# Autodesk Inventor assembly: componentes
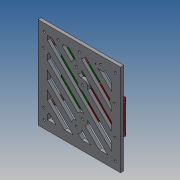
[picture p0: Inventor's stored thumbnail of the model, 180x180]
Saved by Autodesk Inventor 2017 (Build 210142000, 142)
## iProperties
Part Number: componentes
Material: Genérico
Document SubType Name: Assembly
Designer: FABLAB
Author: FABLAB
## Documents named in this file (6)
- C:\Users\Leo\Documents\GitHub\actor-re-actor\models\inventor-caja\Piezas\componentes.iam
- C:\Users\Leo\Documents\GitHub\actor-re-actor\models\inventor-caja\Case\bandeja componentes.ipt
- C:\Users\Leo\Documents\GitHub\actor-re-actor\models\inventor-caja\Piezas\driver motor.ipt
- C:\Users\Leo\Documents\GitHub\actor-re-actor\models\inventor-caja\Piezas\dimmer.ipt
- C:\Users\Leo\Documents\GitHub\actor-re-actor\models\inventor-caja\Piezas\espaciador dimmer.ipt
- C:\Users\Leo\Documents\GitHub\actor-re-actor\models\inventor-caja\Piezas\espaciador driver.ipt
## Components (11 placed, 5 different names)
1. bandeja componentes:1 — Coincidencia:1, Nivelación:1, Coincidencia:3
2. driver motor:1 — Nivelación:1, Nivelación:2, Coincidencia:2, Nivelación:3, Insertar:5, Insertar:6, Insertar:7, Insertar:8
3. dimmer:1 — Coincidencia:2, Nivelación:3, Insertar:1, Insertar:2, Insertar:3, Insertar:4
4. espaciador dimmer:1 — Insertar:3
5. espaciador dimmer:2 — Insertar:4
6. espaciador dimmer:3 — Insertar:2, Coincidencia:3
7. espaciador dimmer:4 — Insertar:1
8. espaciador driver:1 — Insertar:5, Coincidencia:1
9. espaciador driver:2 — Insertar:8
10. espaciador driver:3 — Insertar:6
11. espaciador driver:4 — Insertar:7
## Relationships (14: Insert 8, Mate 3, Flush 3)
- Coincidencia:1 [Mate]: bandeja componentes:1 ↔ espaciador driver:1
- Nivelación:1 [Flush] (4 mm): bandeja componentes:1 ↔ driver motor:1
- Nivelación:2 [Flush] (3 mm): driver motor:1
- Coincidencia:2 [Mate] (2 mm): driver motor:1 ↔ dimmer:1
- Nivelación:3 [Flush] (14 mm): driver motor:1 ↔ dimmer:1
- Coincidencia:3 [Mate]: bandeja componentes:1 ↔ espaciador dimmer:3
- Insertar:1: dimmer:1 ↔ espaciador dimmer:4
- Insertar:2: dimmer:1 ↔ espaciador dimmer:3
- Insertar:3: dimmer:1 ↔ espaciador dimmer:1
- Insertar:4: dimmer:1 ↔ espaciador dimmer:2
- Insertar:5: driver motor:1 ↔ espaciador driver:1
- Insertar:6: driver motor:1 ↔ espaciador driver:3
- Insertar:7: driver motor:1 ↔ espaciador driver:4
- Insertar:8: driver motor:1 ↔ espaciador driver:2
